# Autodesk Inventor assembly: Chasis
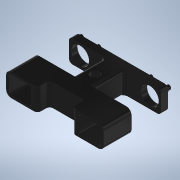
[picture p0: Inventor's stored thumbnail of the model, 180x180]
Saved by Autodesk Inventor 2022 (Build 260153000, 153)
## iProperties
Created: 2021-11-24
Part Number: Chasis
Document SubType Name: Assembly
Designer: JK
Author: JK
## Documents named in this file (3)
- C:\Users\JK\Documents\Inventor\N20 Leg Actuator\N20-Leg-Actuator\CADfiles\Chasis.iam
- C:\Users\JK\Documents\Inventor\N20 Leg Actuator\N20-Leg-Actuator\CADfiles\Base.ipt
- C:\Users\JK\Documents\Inventor\N20 Leg Actuator\N20-Leg-Actuator\CADfiles\PotHolder.ipt
## Components (2 placed, 2 different names)
1. Base:1
2. PotHolder:1
## Relationships (2: Angle 1, Mate 1)
- [Angle] (0 deg): Base:1 ↔ PotHolder:1
- [Mate]: Base:1 ↔ PotHolder:1
